# Autodesk Inventor assembly: Gantry Assembly
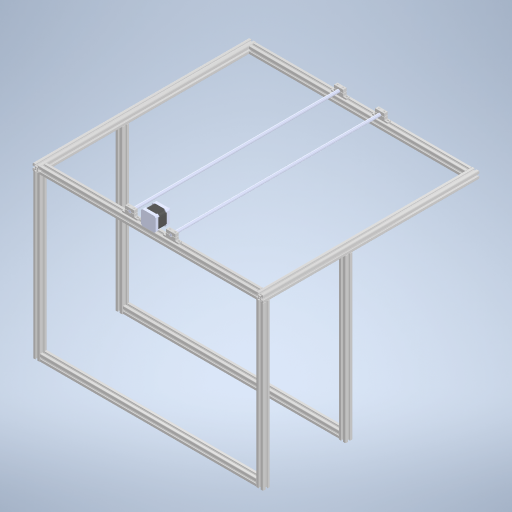
[picture p0: Inventor's stored thumbnail of the model, 512x512]
Saved by Autodesk Inventor 2023 (Build 270158000, 158)
## iProperties
Created: 2023-01-25
Part Number: Gantry Assembly
Document SubType Name: Assembly
Designer: Steven
Author: Steven
## Documents named in this file (14)
- C:\Users\steve\OneDrive\Documents\McMaster University\Courses-Year5\4TB6 Capstone Design Project\The_Nursery_Project\parts\Tray Dropper\Gantry\Gantry Assembly.iam
- C:\Users\steve\Downloads\5537T012_T-Slotted Framing - 1.5ft.ipt
- C:\Users\steve\Downloads\5537T751_T-Slotted Framing - 2ft.ipt
- C:\Users\steve\Downloads\nema-17-41.snapshot.2\Nema 17 stepper.ipt
- C:\Users\steve\Downloads\5537T012_T-Slotted Framing - 1.5ft1.ipt
- C:\Users\steve\Downloads\5537T012_T-Slotted Framing - 1.5ft2.ipt
- C:\Users\steve\Downloads\5537T012_T-Slotted Framing - 1.5ft11.ipt
- C:\Users\steve\Downloads\5537T751_T-Slotted Framing - 2ft1.ipt
- C:\Users\steve\Downloads\5537T751_T-Slotted Framing - 2ft11.ipt
- C:\Users\steve\OneDrive\Documents\McMaster University\Courses-Year5\4TB6 Capstone Design Project\The_Nursery_Project\parts\Tray Dropper\Gantry\5537T751_T-Slotted Framing - 2ft.ipt
- C:\Users\steve\OneDrive\Documents\McMaster University\Courses-Year5\4TB6 Capstone Design Project\The_Nursery_Project\parts\Tray Dropper\Gantry\5537T751_T-Slotted Framing - 2ft1.ipt
- C:\Users\steve\Downloads\5537T751_T-Slotted Framing - 2ft2.ipt
- C:\Users\steve\OneDrive\Documents\McMaster University\Courses-Year5\4TB6 Capstone Design Project\The_Nursery_Project\parts\Tray Dropper\Gantry\1865K21_Easy-Access Base-Mounted Shaft Support.ipt
- C:\Users\steve\OneDrive\Documents\McMaster University\Courses-Year5\4TB6 Capstone Design Project\The_Nursery_Project\parts\Tray Dropper\Gantry\6112K46_Linear Motion Shaft.ipt
## Components (17 placed, 11 different names)
1. 5537T012_T-Slotted Framing - 1.5ft:1 — Mate:12, Flush:15, Mate:17, Flush:20, Flush:21, Flush:23, Mate:18
2. Nema 17 stepper:1 — Flush:12, Mate:26, Flush:33
3. 5537T751_T-Slotted Framing - 2ft:1 — Flush:12, Mate:12, Flush:15, Flush:22, Mate:19, Flush:24, Mate:20, Flush:25, Mate:26, Flush:33
4. 5537T012_T-Slotted Framing - 1.5ft1:1
5. 5537T012_T-Slotted Framing - 1.5ft2:1
6. 5537T012_T-Slotted Framing - 1.5ft11:1
7. 5537T751_T-Slotted Framing - 2ft1:1 — Mate:17, Flush:20, Flush:21
8. 5537T751_T-Slotted Framing - 2ft11:1
9. 5537T751_T-Slotted Framing - 2ft:2 — Flush:22, Flush:23, Mate:18
10. 5537T751_T-Slotted Framing - 2ft1:2
11. 5537T751_T-Slotted Framing - 2ft2:1 — Mate:21, Flush:26, Mate:22, Flush:27
12. 1865K21_Easy-Access Base-Mounted Shaft Support:1 — Mate:19, Flush:24, Flush:28, Mate:23, Flush:29
13. 1865K21_Easy-Access Base-Mounted Shaft Support:2 — Mate:20, Flush:25, Flush:30, Flush:31, Mate:25
14. 1865K21_Easy-Access Base-Mounted Shaft Support:3 — Mate:21, Flush:26, Mate:24
15. 1865K21_Easy-Access Base-Mounted Shaft Support:4 — Mate:22, Flush:27, Flush:32
16. 6112K46_Linear Motion Shaft:1 — Flush:28, Mate:23, Flush:29, Mate:24
17. 6112K46_Linear Motion Shaft:2 — Flush:30, Flush:31, Mate:25, Flush:32
## Relationships (27: Flush 16, Mate 11)
- Flush:12: Nema 17 stepper:1 ↔ 5537T751_T-Slotted Framing - 2ft:1
- Mate:12: 5537T012_T-Slotted Framing - 1.5ft:1 ↔ 5537T751_T-Slotted Framing - 2ft:1
- Flush:15: 5537T012_T-Slotted Framing - 1.5ft:1 ↔ 5537T751_T-Slotted Framing - 2ft:1
- Mate:17: 5537T012_T-Slotted Framing - 1.5ft:1 ↔ 5537T751_T-Slotted Framing - 2ft1:1
- Flush:20: 5537T012_T-Slotted Framing - 1.5ft:1 ↔ 5537T751_T-Slotted Framing - 2ft1:1
- Flush:21: 5537T012_T-Slotted Framing - 1.5ft:1 ↔ 5537T751_T-Slotted Framing - 2ft1:1
- Flush:22: 5537T751_T-Slotted Framing - 2ft:1 ↔ 5537T751_T-Slotted Framing - 2ft:2
- Flush:23: 5537T012_T-Slotted Framing - 1.5ft:1 ↔ 5537T751_T-Slotted Framing - 2ft:2
- Mate:18: 5537T012_T-Slotted Framing - 1.5ft:1 ↔ 5537T751_T-Slotted Framing - 2ft:2
- Mate:19: 5537T751_T-Slotted Framing - 2ft:1 ↔ 1865K21_Easy-Access Base-Mounted Shaft Support:1
- Flush:24 (-5 mm): 5537T751_T-Slotted Framing - 2ft:1 ↔ 1865K21_Easy-Access Base-Mounted Shaft Support:1
- Mate:20: 5537T751_T-Slotted Framing - 2ft:1 ↔ 1865K21_Easy-Access Base-Mounted Shaft Support:2
- Flush:25 (5 mm): 5537T751_T-Slotted Framing - 2ft:1 ↔ 1865K21_Easy-Access Base-Mounted Shaft Support:2
- Mate:21: 5537T751_T-Slotted Framing - 2ft2:1 ↔ 1865K21_Easy-Access Base-Mounted Shaft Support:3
- Flush:26 (5 mm): 5537T751_T-Slotted Framing - 2ft2:1 ↔ 1865K21_Easy-Access Base-Mounted Shaft Support:3
- Mate:22: 5537T751_T-Slotted Framing - 2ft2:1 ↔ 1865K21_Easy-Access Base-Mounted Shaft Support:4
- Flush:27 (5 mm): 5537T751_T-Slotted Framing - 2ft2:1 ↔ 1865K21_Easy-Access Base-Mounted Shaft Support:4
- Flush:28: 1865K21_Easy-Access Base-Mounted Shaft Support:1 ↔ 6112K46_Linear Motion Shaft:1
- Mate:23: 1865K21_Easy-Access Base-Mounted Shaft Support:1 ↔ 6112K46_Linear Motion Shaft:1
- Flush:29 (-12.192 mm): 1865K21_Easy-Access Base-Mounted Shaft Support:1 ↔ 6112K46_Linear Motion Shaft:1
- Mate:24: 1865K21_Easy-Access Base-Mounted Shaft Support:3 ↔ 6112K46_Linear Motion Shaft:1
- Flush:30: 1865K21_Easy-Access Base-Mounted Shaft Support:2 ↔ 6112K46_Linear Motion Shaft:2
- Flush:31: 1865K21_Easy-Access Base-Mounted Shaft Support:2 ↔ 6112K46_Linear Motion Shaft:2
- Mate:25 (12.192 mm): 1865K21_Easy-Access Base-Mounted Shaft Support:2 ↔ 6112K46_Linear Motion Shaft:2
- Flush:32: 1865K21_Easy-Access Base-Mounted Shaft Support:4 ↔ 6112K46_Linear Motion Shaft:2
- Mate:26: Nema 17 stepper:1 ↔ 5537T751_T-Slotted Framing - 2ft:1
- Flush:33: Nema 17 stepper:1 ↔ 5537T751_T-Slotted Framing - 2ft:1
